# Autodesk Inventor assembly: RotatingCamera
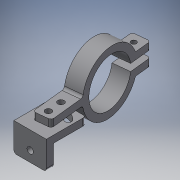
[picture p0: Inventor's stored thumbnail of the model, 180x180]
Saved by Autodesk Inventor 2019 (Build 230136000, 136)
## iProperties
Created: 2019-08-13
Part Number: RotatingCamera
Document SubType Name: Assembly
Designer: aorfi
Author: aorfi
## Documents named in this file (3)
- C:\Users\aorfi\Documents\IQC\CustomParts\RotatingCamera.iam
- C:\Users\aorfi\Documents\IQC\CustomParts\CameraClampRotate.ipt
- C:\Users\aorfi\Documents\IQC\CustomParts\RotateLBracket.ipt
## Components (2 placed, 2 different names)
1. CameraClampRotate:1 — Mate:2, Mate:3
2. RotateLBracket:1 — Flush:1, Flush:2, Flush:3, Mate:2, Mate:3
## Relationships (5: Flush 3, Mate 2)
- Flush:1: RotateLBracket:1
- Flush:2: RotateLBracket:1
- Flush:3: RotateLBracket:1
- Mate:2: CameraClampRotate:1 ↔ RotateLBracket:1
- Mate:3: CameraClampRotate:1 ↔ RotateLBracket:1
